# Autodesk Inventor assembly: Assembly4
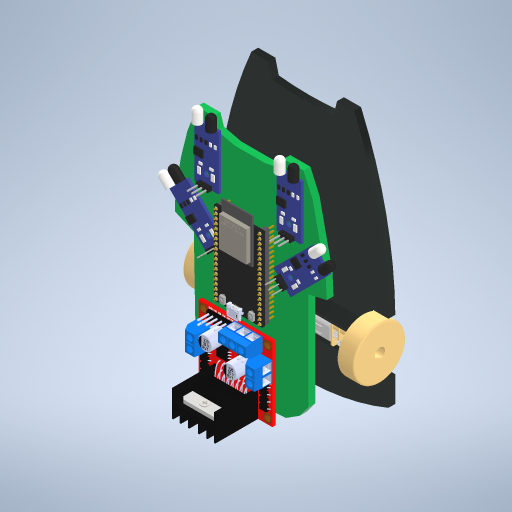
[picture p0: Inventor's stored thumbnail of the model, 512x512]
Saved by Autodesk Inventor 2024 (Build 280153000, 153)
## iProperties
Created: 2024-04-14
Part Number: Assembly4
Document SubType Name: Assembly
Designer: Hitesh
Author: Hitesh
## Documents named in this file (7)
- C:\Users\Hitesh\Documents\Inventor\Mickey\Assembly4.iam
- C:\Users\Hitesh\Documents\Inventor\Mickey\Part2.ipt
- C:\Users\Hitesh\Documents\Inventor\Mickey\Infrared Obstacle Detecting Module v4.iam
- C:\Users\Hitesh\Documents\Inventor\Mickey\ESP32-WROOM-32D-Assembly.iam
- C:\Users\Hitesh\Documents\Inventor\Mickey\L298N Driver DC Motor, Stepper Motor.ipt
- C:\Users\Hitesh\Documents\Inventor\Mickey\Part1.ipt
- C:\Users\Hitesh\Documents\Inventor\Mickey\N20 Mini Micro Metall Gear Motor DC 3-6-12V v1.ipt
## Components (10 placed, 6 different names)
1. Part2:1 — Mate:1, Mate:2, Mate:3, Mate:4, Flush:1, Mate:5, Flush:2, Mate:6, Mate:7, Flush:3, Mate:8, Mate:10, Mate:12, Mate:14
2. Infrared Obstacle Detecting Module v4:1 [sub-assembly] — Mate:3, Angle:2, Mate:10, Mate:11
3. Infrared Obstacle Detecting Module v4:2 [sub-assembly] — Mate:1, Flush:2, Mate:6, Flush:4
4. Infrared Obstacle Detecting Module v4:3 [sub-assembly] — Mate:4, Angle:1, Mate:8, Mate:9
5. Infrared Obstacle Detecting Module v4:4 [sub-assembly] — Mate:2, Flush:1, Mate:5
6. ESP32-WROOM-32D-Assembly:1 [sub-assembly] — Mate:7, Flush:3, Flush:4, Angle:1, Mate:9, Angle:2, Mate:11, Mate:13, Flush:5, Flush:6
7. L298N Driver DC Motor, Stepper Motor:1 — Mate:12, Mate:13, Flush:5, Flush:7
8. Part1:1 — Mate:14, Flush:6, Flush:7, Mate:15, Mate:16, Mate:17, Mate:18, Mate:19, Mate:20
9. N20 Mini Micro Metall Gear Motor DC 3-6-12V v1:1 — Mate:15, Mate:16, Mate:17
10. N20 Mini Micro Metall Gear Motor DC 3-6-12V v1:2 — Mate:18, Mate:19, Mate:20
## Relationships (29: Mate 20, Flush 7, Angle 2)
- Mate:1: Part2:1 ↔ Infrared Obstacle Detecting Module v4:2
- Mate:2: Part2:1 ↔ Infrared Obstacle Detecting Module v4:4
- Mate:3: Part2:1 ↔ Infrared Obstacle Detecting Module v4:1
- Mate:4: Part2:1 ↔ Infrared Obstacle Detecting Module v4:3
- Flush:1 (5.08 mm): Part2:1 ↔ Infrared Obstacle Detecting Module v4:4
- Mate:5 (5.08 mm): Part2:1 ↔ Infrared Obstacle Detecting Module v4:4
- Flush:2 (5.08 mm): Part2:1 ↔ Infrared Obstacle Detecting Module v4:2
- Mate:6 (5.08 mm): Part2:1 ↔ Infrared Obstacle Detecting Module v4:2
- Mate:7 (6.35 mm): Part2:1 ↔ ESP32-WROOM-32D-Assembly:1
- Flush:3 (-19.05 mm): Part2:1 ↔ ESP32-WROOM-32D-Assembly:1
- Flush:4 (17.78 mm): Infrared Obstacle Detecting Module v4:2 ↔ ESP32-WROOM-32D-Assembly:1
- Angle:1 (45 deg): Infrared Obstacle Detecting Module v4:3 ↔ ESP32-WROOM-32D-Assembly:1
- Mate:8 (2.54 mm): Part2:1 ↔ Infrared Obstacle Detecting Module v4:3
- Mate:9 (10.16 mm): Infrared Obstacle Detecting Module v4:3 ↔ ESP32-WROOM-32D-Assembly:1
- Angle:2 (-45 deg): Infrared Obstacle Detecting Module v4:1 ↔ ESP32-WROOM-32D-Assembly:1
- Mate:10 (2.54 mm): Part2:1 ↔ Infrared Obstacle Detecting Module v4:1
- Mate:11 (10.16 mm): Infrared Obstacle Detecting Module v4:1 ↔ ESP32-WROOM-32D-Assembly:1
- Mate:12 (7.62 mm): Part2:1 ↔ L298N Driver DC Motor, Stepper Motor:1
- Mate:13 (2.54 mm): ESP32-WROOM-32D-Assembly:1 ↔ L298N Driver DC Motor, Stepper Motor:1
- Flush:5 (-7.62 mm): ESP32-WROOM-32D-Assembly:1 ↔ L298N Driver DC Motor, Stepper Motor:1
- Mate:14 (25.4 mm): Part2:1 ↔ Part1:1
- Flush:6 (50.8 mm): ESP32-WROOM-32D-Assembly:1 ↔ Part1:1
- Flush:7 (21.336 mm): L298N Driver DC Motor, Stepper Motor:1 ↔ Part1:1
- Mate:15: Part1:1 ↔ N20 Mini Micro Metall Gear Motor DC 3-6-12V v1:1
- Mate:16: Part1:1 ↔ N20 Mini Micro Metall Gear Motor DC 3-6-12V v1:1
- Mate:17: Part1:1 ↔ N20 Mini Micro Metall Gear Motor DC 3-6-12V v1:1
- Mate:18: Part1:1 ↔ N20 Mini Micro Metall Gear Motor DC 3-6-12V v1:2
- Mate:19: Part1:1 ↔ N20 Mini Micro Metall Gear Motor DC 3-6-12V v1:2
- Mate:20: Part1:1 ↔ N20 Mini Micro Metall Gear Motor DC 3-6-12V v1:2
